# Autodesk Inventor assembly: Montagem
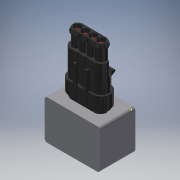
[picture p0: Inventor's stored thumbnail of the model, 180x180]
Saved by Autodesk Inventor 2019 (Build 230136000, 136)
## iProperties
Created: 2021-05-27
Part Number: Montagem
Document SubType Name: Assembly
Designer: hoope
Author: hoope
## Documents named in this file (5)
- C:\Users\hoope\OneDrive\Documentos\Lucas\Faculdade\BAJA\Inventor\Atividades\Nova fixação do acelerometro 2\Montagem.iam
- C:\Users\hoope\OneDrive\Documentos\Lucas\Faculdade\BAJA\Inventor\Atividades\Nova fixação do acelerometro 2\Caixa.ipt
- C:\Users\hoope\OneDrive\Documentos\Lucas\Faculdade\BAJA\Inventor\Atividades\Nova fixação do acelerometro 2\MPU6050.ipt
- C:\Users\hoope\OneDrive\Documentos\Lucas\Faculdade\BAJA\Inventor\Atividades\Nova fixação do acelerometro 2\AMP 4 position.ipt
- C:\Users\hoope\OneDrive\Documentos\Lucas\Faculdade\BAJA\Inventor\Atividades\Nova fixação do acelerometro 2\Tampa.ipt
## Components (4 placed, 4 different names)
1. Caixa:1 — Coincidência:1, Coincidência:2, Coincidência:3, Coincidência:4, Coincidência:5, Coincidência:6, Coincidência:7, Coincidência:8
2. MPU6050:1 — Coincidência:1, Coincidência:2
3. AMP 4 position:1 — Coincidência:3, Coincidência:4, Coincidência:5
4. Tampa:1 — Coincidência:6, Coincidência:7, Coincidência:8
## Relationships (8: Mate 8)
- Coincidência:1 [Mate]: Caixa:1 ↔ MPU6050:1
- Coincidência:2 [Mate]: Caixa:1 ↔ MPU6050:1
- Coincidência:3 [Mate]: Caixa:1 ↔ AMP 4 position:1
- Coincidência:4 [Mate]: Caixa:1 ↔ AMP 4 position:1
- Coincidência:5 [Mate]: Caixa:1 ↔ AMP 4 position:1
- Coincidência:6 [Mate]: Caixa:1 ↔ Tampa:1
- Coincidência:7 [Mate]: Caixa:1 ↔ Tampa:1
- Coincidência:8 [Mate]: Caixa:1 ↔ Tampa:1
